# Autodesk Inventor assembly: assembly_try1
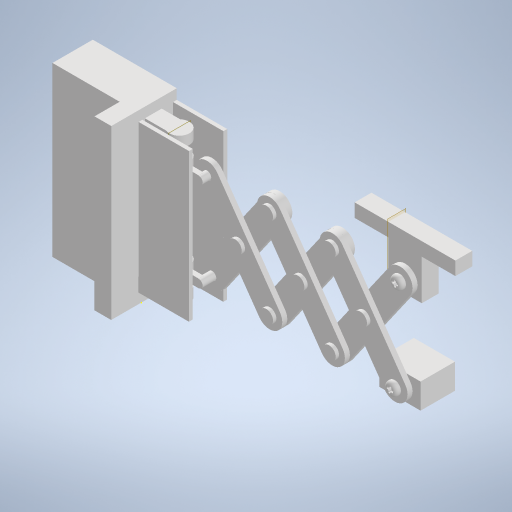
[picture p0: Inventor's stored thumbnail of the model, 512x512]
Saved by Autodesk Inventor 2024 (Build 280153000, 153)
## iProperties
Created: 2024-02-29
Part Number: assembly_try1
Document SubType Name: Assembly
Designer: clbri
Author: clbri
## Documents named in this file (12)
- C:\Users\clbri\Downloads\assembly_try1.iam
- C:\Users\clbri\Downloads\saanvi\top_bracket.ipt
- C:\Users\clbri\Downloads\saanvi\DP3_linkage_extruded.ipt
- C:\Users\clbri\Downloads\saanvi\Team5_screw.ipt
- C:\Users\clbri\Downloads\saanvi\bracket_bottom1.ipt
- C:\Users\clbri\Downloads\saanvi\linkage_bolt_nut.ipt
- C:\Users\clbri\Downloads\saanvi\link_nut_bolt_end.ipt
- C:\Users\clbri\Downloads\saanvi\link_end_fixation.ipt
- C:\Users\clbri\Downloads\saanvi\guide_rod.ipt
- C:\Users\clbri\Downloads\saanvi\link_end_fixation_extended.ipt
- C:\Users\clbri\Downloads\saanvi\rod_end_fixation.ipt
- C:\Users\clbri\Downloads\saanvi\guided hand 2.ipt
## Components (32 placed, 11 different names)
1. top_bracket:1 — Mate:1, Mate:2, Flush:1
2. DP3_linkage_extruded:1 — Mate:1, Mate:2, Mate:3, Mate:4, Mate:5, Mate:6, Mate:11, Mate:12, Mate:24, Mate:48, Mate:49
3. DP3_linkage_extruded:2 — Mate:14, Mate:15, Mate:17, Mate:22, Mate:25, Mate:28, Mate:30, Mate:32, Mate:34, Angle:4, Angle:5
4. DP3_linkage_extruded:3 — Mate:15, Mate:16, Mate:18, Mate:21, Mate:25, Mate:27, Mate:45, Mate:46, Mate:47, Angle:4, Angle:5
5. DP3_linkage_extruded:4 — Mate:5, Mate:6, Mate:7, Mate:9, Mate:10, Mate:13, Mate:24, Mate:27, Mate:29, Mate:35
6. DP3_linkage_extruded:5 — Mate:17, Mate:19, Mate:23, Mate:26, Mate:28, Mate:37, Mate:39, Mate:56, Mate:60, Angle:3
7. DP3_linkage_extruded:6 — Mate:18, Mate:19, Mate:20, Mate:26, Mate:31, Mate:33, Mate:50, Mate:55, Angle:3
8. Team5_screw:1 — Mate:8, Mate:9
9. Team5_screw:2 — Mate:3, Mate:4
10. bracket_bottom1:1 — Mate:7, Mate:8, Mate:10, Flush:1
11. linkage_bolt_nut:1 — Mate:22, Mate:32, Mate:36
12. linkage_bolt_nut:2 — Mate:23, Mate:31, Mate:38
13. linkage_bolt_nut:6 — Mate:21, Mate:30, Mate:43
14. linkage_bolt_nut:7 — Mate:20, Mate:33, Mate:40
15. linkage_bolt_nut:8 — Mate:11, Mate:35, Mate:42
16. linkage_bolt_nut:9 — Mate:13, Mate:16, Mate:29, Mate:44
17. linkage_bolt_nut:10 — Mate:12, Mate:14, Mate:34, Mate:41
18. link_nut_bolt_end:2 — Mate:38, Mate:39
19. link_nut_bolt_end:3 — Mate:44, Mate:45
20. link_nut_bolt_end:4 — Mate:42, Mate:48
21. link_nut_bolt_end:5 — Mate:43, Mate:46
22. link_nut_bolt_end:6 — Mate:40, Mate:47
23. link_nut_bolt_end:7 — Mate:41, Mate:49
24. link_nut_bolt_end:8 — Mate:36, Mate:37
25. link_end_fixation:1 — Mate:50, Mate:52, Mate:54, Flush:2, Mate:57, Angle:1, Mate:66
26. link_nut_bolt_end:9 — Mate:56, Mate:59
27. link_nut_bolt_end:10 — Mate:52, Mate:54, Mate:55, Flush:2
28. guide_rod:1 — Mate:57, Mate:58, Mate:61, Mate:62, Mate:63, Mate:64
29. link_end_fixation_extended:1 — Mate:58, Mate:59, Mate:60, Angle:2, Mate:65
30. rod_end_fixation:1 — Mate:61, Mate:62, Angle:1, Mate:66, Mate:67, Mate:68, Mate:69
31. rod_end_fixation:2 — Mate:63, Mate:64, Angle:2, Mate:65
32. guided hand 2:1 — Mate:67, Mate:68, Mate:69
## Relationships (74: Mate 67, Angle 5, Flush 2)
- Mate:1: top_bracket:1 ↔ DP3_linkage_extruded:1
- Mate:2: top_bracket:1 ↔ DP3_linkage_extruded:1
- Mate:3: DP3_linkage_extruded:1 ↔ Team5_screw:2
- Mate:4: DP3_linkage_extruded:1 ↔ Team5_screw:2
- Mate:5: DP3_linkage_extruded:1 ↔ DP3_linkage_extruded:4
- Mate:6: DP3_linkage_extruded:1 ↔ DP3_linkage_extruded:4
- Mate:7: DP3_linkage_extruded:4 ↔ bracket_bottom1:1
- Mate:8: Team5_screw:1 ↔ bracket_bottom1:1
- Mate:9: DP3_linkage_extruded:4 ↔ Team5_screw:1
- Mate:10: DP3_linkage_extruded:4 ↔ bracket_bottom1:1
- Mate:11: DP3_linkage_extruded:1 ↔ linkage_bolt_nut:8
- Mate:12: DP3_linkage_extruded:1 ↔ linkage_bolt_nut:10
- Mate:13: DP3_linkage_extruded:4 ↔ linkage_bolt_nut:9
- Flush:1 (2.25 mm): top_bracket:1 ↔ bracket_bottom1:1
- Mate:14: DP3_linkage_extruded:2 ↔ linkage_bolt_nut:10
- Mate:15: DP3_linkage_extruded:2 ↔ DP3_linkage_extruded:3
- Mate:16: DP3_linkage_extruded:3 ↔ linkage_bolt_nut:9
- Mate:17: DP3_linkage_extruded:2 ↔ DP3_linkage_extruded:5
- Mate:18: DP3_linkage_extruded:3 ↔ DP3_linkage_extruded:6
- Mate:19: DP3_linkage_extruded:5 ↔ DP3_linkage_extruded:6
- Mate:20: DP3_linkage_extruded:6 ↔ linkage_bolt_nut:7
- Mate:21: DP3_linkage_extruded:3 ↔ linkage_bolt_nut:6
- Mate:22: DP3_linkage_extruded:2 ↔ linkage_bolt_nut:1
- Mate:23: DP3_linkage_extruded:5 ↔ linkage_bolt_nut:2
- Mate:24: DP3_linkage_extruded:1 ↔ DP3_linkage_extruded:4
- Mate:25: DP3_linkage_extruded:2 ↔ DP3_linkage_extruded:3
- Mate:26: DP3_linkage_extruded:5 ↔ DP3_linkage_extruded:6
- Mate:27: DP3_linkage_extruded:3 ↔ DP3_linkage_extruded:4
- Mate:28: DP3_linkage_extruded:2 ↔ DP3_linkage_extruded:5
- Mate:29: DP3_linkage_extruded:4 ↔ linkage_bolt_nut:9
- Mate:30: DP3_linkage_extruded:2 ↔ linkage_bolt_nut:6
- Mate:31: DP3_linkage_extruded:6 ↔ linkage_bolt_nut:2
- Mate:32: DP3_linkage_extruded:2 ↔ linkage_bolt_nut:1
- Mate:33: DP3_linkage_extruded:6 ↔ linkage_bolt_nut:7
- Mate:34: DP3_linkage_extruded:2 ↔ linkage_bolt_nut:10
- Mate:35: DP3_linkage_extruded:4 ↔ linkage_bolt_nut:8
- Mate:36: linkage_bolt_nut:1 ↔ link_nut_bolt_end:8
- Mate:37: DP3_linkage_extruded:5 ↔ link_nut_bolt_end:8
- Mate:38: linkage_bolt_nut:2 ↔ link_nut_bolt_end:2
- Mate:39: DP3_linkage_extruded:5 ↔ link_nut_bolt_end:2
- Mate:40: linkage_bolt_nut:7 ↔ link_nut_bolt_end:6
- Mate:41: linkage_bolt_nut:10 ↔ link_nut_bolt_end:7
- Mate:42: linkage_bolt_nut:8 ↔ link_nut_bolt_end:4
- Mate:43: linkage_bolt_nut:6 ↔ link_nut_bolt_end:5
- Mate:44: linkage_bolt_nut:9 ↔ link_nut_bolt_end:3
- Mate:45: DP3_linkage_extruded:3 ↔ link_nut_bolt_end:3
- Mate:46: DP3_linkage_extruded:3 ↔ link_nut_bolt_end:5
- Mate:47: DP3_linkage_extruded:3 ↔ link_nut_bolt_end:6
- Mate:48: DP3_linkage_extruded:1 ↔ link_nut_bolt_end:4
- Mate:49: DP3_linkage_extruded:1 ↔ link_nut_bolt_end:7
- Mate:50: DP3_linkage_extruded:6 ↔ link_end_fixation:1
- Mate:52: link_end_fixation:1 ↔ link_nut_bolt_end:10
- Mate:54: link_end_fixation:1 ↔ link_nut_bolt_end:10
- Mate:55: DP3_linkage_extruded:6 ↔ link_nut_bolt_end:10
- Flush:2: link_end_fixation:1 ↔ link_nut_bolt_end:10
- Mate:56: DP3_linkage_extruded:5 ↔ link_nut_bolt_end:9
- Mate:57: link_end_fixation:1 ↔ guide_rod:1
- Mate:58: guide_rod:1 ↔ link_end_fixation_extended:1
- Mate:59: link_nut_bolt_end:9 ↔ link_end_fixation_extended:1
- Mate:60: DP3_linkage_extruded:5 ↔ link_end_fixation_extended:1
- Mate:61: guide_rod:1 ↔ rod_end_fixation:1
- Mate:62: guide_rod:1 ↔ rod_end_fixation:1
- Mate:63: guide_rod:1 ↔ rod_end_fixation:2
- Mate:64: guide_rod:1 ↔ rod_end_fixation:2
- Angle:1 (180 deg): link_end_fixation:1 ↔ rod_end_fixation:1
- Angle:2 (0 deg): link_end_fixation_extended:1 ↔ rod_end_fixation:2
- Mate:65: link_end_fixation_extended:1 ↔ rod_end_fixation:2
- Mate:66: link_end_fixation:1 ↔ rod_end_fixation:1
- Mate:67: rod_end_fixation:1 ↔ guided hand 2:1
- Mate:68: rod_end_fixation:1 ↔ guided hand 2:1
- Mate:69 (40 mm): rod_end_fixation:1 ↔ guided hand 2:1
- Angle:3 (0 deg): DP3_linkage_extruded:5 ↔ DP3_linkage_extruded:6
- Angle:4 (0 deg): DP3_linkage_extruded:2 ↔ DP3_linkage_extruded:3
- Angle:5 (0 deg): DP3_linkage_extruded:2 ↔ DP3_linkage_extruded:3
